# Autodesk Inventor assembly: PCB_LIHU
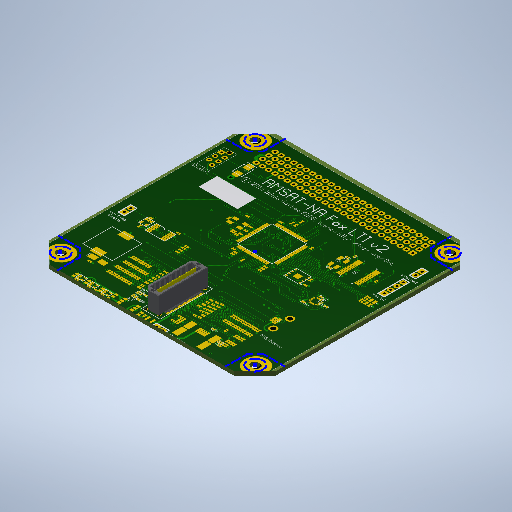
[picture p0: Inventor's stored thumbnail of the model, 512x512]
Saved by Autodesk Inventor 2025 (Build 290162000, 162)
## iProperties
Created: 2011-10-12
Part Number: PCB_LIHU
Document SubType Name: Assembly
Designer: Robert Davis
Description: TX PCB
Mass: 41.3265 g
Surface Area: 295.326 cm^2
Volume: 17.1094 cm^3
Density: 2.41542 g/cm^3
Author: Robert Davis
## Documents named in this file (4)
- C:\Users\arobi\Documents\Repos\fox-plus\mechanical\AssemblyModels\PCB_LIHU.iam
- C:\Users\arobi\Documents\Repos\fox-plus\structure\3d_models\CommercialFrame\Samtec_QTH-030-02-L-D-A.ipt
- C:\Users\arobi\Documents\Repos\fox-plus\structure\3d_models\CommercialFrame\Samtec_QSH-030-01-L-D-A.ipt
- C:\Users\arobi\Documents\Repos\fox-plus\mechanical\AssemblyModels\PCB_LIHU.ipt
## Components (3 placed, 3 different names)
1. PCB_LIHU:1 — Mate:1, Angle:1, Mate:5, Mate:4
2. Samtec_QTH-030-02-L-D-A:1 — Mate:1, Angle:1
3. Samtec_QSH-030-01-L-D-A:1 — Mate:5, Mate:4
## Relationships (6: Mate 4, Angle 2)
- Mate:1: PCB_LIHU:1 ↔ Samtec_QTH-030-02-L-D-A:1
- [Mate]: PCB_LIHU:1 ↔ Samtec_QTH-030-02-L-D-A:1
- Angle:1 (180 deg): PCB_LIHU:1 ↔ Samtec_QTH-030-02-L-D-A:1
- Mate:5: PCB_LIHU:1 ↔ Samtec_QSH-030-01-L-D-A:1
- Mate:4: PCB_LIHU:1 ↔ Samtec_QSH-030-01-L-D-A:1
- [Angle] (180 deg): PCB_LIHU:1 ↔ Samtec_QSH-030-01-L-D-A:1
